# Autodesk Inventor assembly: Filtro
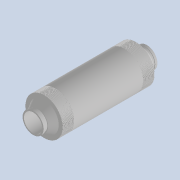
[picture p0: Inventor's stored thumbnail of the model, 180x180]
Saved by Autodesk Inventor 2021 (Build 250183000, 183)
## iProperties
Created: 2021-06-01
Part Number: Filtro
Document SubType Name: Assembly
Designer: Admin
Author: Admin
## Documents named in this file (3)
- E:\Documentos\Documentos\Michael_Rodriguez\Universidad_Nacional\Doceaba matricula\PAI\Proyecto PAI\Proyecto_PAI_2021\01 CAD\Filtro.iam
- E:\Documentos\Documentos\Michael_Rodriguez\Universidad_Nacional\Doceaba matricula\PAI\Proyecto PAI\Proyecto_PAI_2021\01 CAD\CuerpoPrincipal_filtro.ipt
- E:\Documentos\Documentos\Michael_Rodriguez\Universidad_Nacional\Doceaba matricula\PAI\Proyecto PAI\Proyecto_PAI_2021\01 CAD\punta_filtro.ipt
## Components (3 placed, 2 different names)
1. CuerpoPrincipal_filtro:1 — Rígido:1, Rígido:2
2. punta_filtro:1 — Rígido:1
3. punta_filtro:2 — Rígido:2
## Relationships (2: WeldJoint 2)
- Rígido:1 [WeldJoint]: CuerpoPrincipal_filtro:1 ↔ punta_filtro:1
- Rígido:2 [WeldJoint]: CuerpoPrincipal_filtro:1 ↔ punta_filtro:2
